# Autodesk Inventor assembly: kez
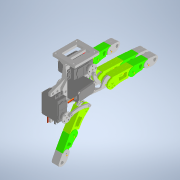
[picture p0: Inventor's stored thumbnail of the model, 180x180]
Saved by Autodesk Inventor 2020 (Build 240168000, 168)
## iProperties
Created: 2019-08-09
Part Number: kez
Document SubType Name: Assembly
Designer: Horváth Patrik
Author: Horváth Patrik
## Documents named in this file (12)
- D:\I.V.A.N\LEGO\INDACT\Robotkéz\kéz12.0\kez.iam
- D:\I.V.A.N\LEGO\INDACT\Robotkéz\kéz12.0\kezfej3.ipt
- D:\I.V.A.N\LEGO\INDACT\Robotkéz\kéz12.0\motor_sima.iam
- D:\I.V.A.N\LEGO\INDACT\Robotkéz\kéz12.0\ujj_alapmodell.iam
- D:\I.V.A.N\LEGO\INDACT\Robotkéz\kéz11.0\INDACTfel2.ipt
- D:\I.V.A.N\LEGO\INDACT\Robotkéz\kéz12.0\motortarcsa.ipt
- D:\I.V.A.N\LEGO\INDACT\Robotkéz\kéz12.0\Part2.ipt
- D:\I.V.A.N\LEGO\INDACT\Robotkéz\kéz12.0\Part3.ipt
- D:\I.V.A.N\LEGO\INDACT\Robotkéz\kéz12.0\Part5.ipt
- C:\Users\Horváth Patrik\Documents\Inventor\Content Center Files\R2020\en-US\ISO 4762(2)\ISO 4762 - M4 x 6ISO.ipt
- C:\Users\Horváth Patrik\Documents\Inventor\Content Center Files\R2020\en-US\ISO 4762(2)\ISO 4762 - M2 x 20ISO.ipt
- D:\I.V.A.N\LEGO\INDACT\Robotkéz\kéz12.0\tarto.ipt
## Components (19 placed, 11 different names)
1. kezfej3:1 — Mate:8, Mate:9, Mate:12, Flush:1, Angle:3, Angle:4, Mate:24, Mate:25, Mate:26, Mate:27, Mate:28, Mate:29, Mate:31, Mate:32, Mate:33, Mate:34, Mate:35, Mate:43, Angle:7, Flush:8, Mate:56, Flush:10, Mate:61, Mate:63, Mate:64, Mate:65
2. motor_sima:1 [sub-assembly] — Mate:30, Mate:31, Flush:3, Mate:38, Mate:53, Mate:54, Angle:8, Mate:59, Mate:60
3. motor_sima:2 [sub-assembly] — Flush:2, Mate:18, Mate:19, Angle:5, Mate:30, Mate:38, Flush:8, Mate:56
4. ujj_alapmodell:1 [sub-assembly] — Angle:3, Mate:23, Angle:9, Mate:58, Mate:63, Mate:64
5. ujj_alapmodell:2 [sub-assembly] — Mate:8, Mate:9, Angle:4, Flush:2, Mate:23
6. INDACTfel2:1 — Mate:12, Flush:1
7. motortarcsa:1 — Mate:18, Mate:19, Angle:5, Angle:9, Flush:9
8. ujj_alapmodell:3 [sub-assembly] — Mate:24, Mate:25, Mate:26, Flush:3, Flush:5
9. ujj_alapmodell:4 [sub-assembly] — Mate:27, Mate:28, Mate:29, Mate:49
10. ujj_alapmodell:5 [sub-assembly] — Mate:32, Mate:33, Mate:34, Flush:4, Mate:47
11. motor_sima:3 [sub-assembly] — Flush:4, Mate:35, Mate:43, Mate:44, Mate:45, Flush:10
12. Part2:1 — Flush:5, Mate:49, Mate:55
13. motortarcsa:3 — Mate:44, Mate:45, Angle:7, Flush:7, Mate:46
14. Part3:1 — Flush:7, Mate:46, Mate:47
15. motortarcsa:4 — Mate:53, Mate:54, Angle:8, Mate:55
16. Part5:1 — Flush:9, Mate:58, Mate:62
17. ISO 4762 M4 x 6:1 — Mate:59, Mate:60
18. ISO 4762 M2 x 20:1 — Mate:61, Mate:62
19. tarto:2 — Mate:65
## Relationships (52: Mate 37, Flush 9, Angle 6)
- Mate:8: kezfej3:1 ↔ ujj_alapmodell:2
- Mate:9: kezfej3:1 ↔ ujj_alapmodell:2
- Mate:12: kezfej3:1 ↔ INDACTfel2:1
- Flush:1: kezfej3:1 ↔ INDACTfel2:1
- Angle:3 (0 deg): kezfej3:1 ↔ ujj_alapmodell:1
- Angle:4 (0 deg): kezfej3:1 ↔ ujj_alapmodell:2
- Flush:2: motor_sima:2 ↔ ujj_alapmodell:2
- Mate:18: motor_sima:2 ↔ motortarcsa:1
- Mate:19: motor_sima:2 ↔ motortarcsa:1
- Angle:5 (0 deg): motor_sima:2 ↔ motortarcsa:1
- Mate:23: ujj_alapmodell:1 ↔ ujj_alapmodell:2
- Mate:24: kezfej3:1 ↔ ujj_alapmodell:3
- Mate:25: kezfej3:1 ↔ ujj_alapmodell:3
- Mate:26: kezfej3:1 ↔ ujj_alapmodell:3
- Mate:27: kezfej3:1 ↔ ujj_alapmodell:4
- Mate:28: kezfej3:1 ↔ ujj_alapmodell:4
- Mate:29: kezfej3:1 ↔ ujj_alapmodell:4
- Mate:30 (1 mm): motor_sima:1 ↔ motor_sima:2
- Mate:31: kezfej3:1 ↔ motor_sima:1
- Flush:3: motor_sima:1 ↔ ujj_alapmodell:3
- Mate:32: kezfej3:1 ↔ ujj_alapmodell:5
- Mate:33: kezfej3:1 ↔ ujj_alapmodell:5
- Mate:34: kezfej3:1 ↔ ujj_alapmodell:5
- Flush:4: ujj_alapmodell:5 ↔ motor_sima:3
- Mate:35: kezfej3:1 ↔ motor_sima:3
- Mate:38 (-20 mm): motor_sima:1 ↔ motor_sima:2
- Mate:43 (10 mm): kezfej3:1 ↔ motor_sima:3
- Flush:5: ujj_alapmodell:3 ↔ Part2:1
- Mate:44: motor_sima:3 ↔ motortarcsa:3
- Mate:45: motor_sima:3 ↔ motortarcsa:3
- Angle:7 (55 deg): kezfej3:1 ↔ motortarcsa:3
- Flush:7: motortarcsa:3 ↔ Part3:1
- Mate:46: motortarcsa:3 ↔ Part3:1
- Mate:47: ujj_alapmodell:5 ↔ Part3:1
- Mate:49: ujj_alapmodell:4 ↔ Part2:1
- Flush:8: kezfej3:1 ↔ motor_sima:2
- Mate:53: motor_sima:1 ↔ motortarcsa:4
- Mate:54: motor_sima:1 ↔ motortarcsa:4
- Angle:8 (50 deg): motor_sima:1 ↔ motortarcsa:4
- Mate:55: Part2:1 ↔ motortarcsa:4
- Mate:56: kezfej3:1 ↔ motor_sima:2
- Angle:9 (0 deg): ujj_alapmodell:1 ↔ motortarcsa:1
- Flush:9: motortarcsa:1 ↔ Part5:1
- Mate:58: ujj_alapmodell:1 ↔ Part5:1
- Flush:10: kezfej3:1 ↔ motor_sima:3
- Mate:59: motor_sima:1 ↔ ISO 4762 M4 x 6:1
- Mate:60: motor_sima:1 ↔ ISO 4762 M4 x 6:1
- Mate:61: kezfej3:1 ↔ ISO 4762 M2 x 20:1
- Mate:62: Part5:1 ↔ ISO 4762 M2 x 20:1
- Mate:63: kezfej3:1 ↔ ujj_alapmodell:1
- Mate:64: kezfej3:1 ↔ ujj_alapmodell:1
- Mate:65: kezfej3:1 ↔ tarto:2
